# Autodesk Inventor assembly: panelsWithKerf
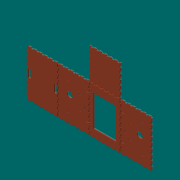
[picture p0: Inventor's stored thumbnail of the model, 180x180]
Saved by Autodesk Inventor 2016 SP2 (Build 200236200, 236)
## iProperties
Created: 2016-09-07
Part Number: panelsWithKerf
Document SubType Name: Assembly
Designer: sawaiz
Author: sawaiz
## Documents named in this file (8)
- C:\Users\sawaiz\OneDrive\projects\splitFlapDisplay\panelsWithKerf.iam
- C:\Users\sawaiz\oneDrive\projects\splitFlapDisplay\frame\front.ipt
- C:\Users\sawaiz\oneDrive\projects\splitFlapDisplay\frame\topBottomPanel.ipt
- C:\Users\sawaiz\oneDrive\projects\splitFlapDisplay\frame\leftSide.ipt
- C:\Users\sawaiz\oneDrive\projects\splitFlapDisplay\frame\rightSide.ipt
- C:\Users\sawaiz\oneDrive\projects\splitFlapDisplay\frame\back.ipt
- C:\Users\sawaiz\oneDrive\projects\splitFlapDisplay\panelsWithKerf.ipt
- C:\Users\sawaiz\OneDrive\projects\splitFlapDisplay\parameters.xlsx
## Components (6 placed, 6 different names)
1. front:1 — Flush:1, Flush:2, Flush:3, Flush:4, Flush:5, Flush:6, Flush:7, Flush:9, Mate:2, Mate:3, Mate:4
2. topBottomPanel:1 — Flush:3, Flush:5, Mate:3
3. leftSide:1 — Flush:2, Flush:7, Flush:8, Mate:1, Mate:2
4. rightSide:1 — Flush:4, Flush:6, Mate:4
5. back:1 — Flush:1, Flush:8, Mate:1
6. panelsWithKerf:1 — Flush:9
## Relationships (13: Flush 9, Mate 4)
- Flush:1: front:1 ↔ back:1
- Flush:2: front:1 ↔ leftSide:1
- Flush:3: front:1 ↔ topBottomPanel:1
- Flush:4: front:1 ↔ rightSide:1
- Flush:5: front:1 ↔ topBottomPanel:1
- Flush:6: front:1 ↔ rightSide:1
- Flush:7: front:1 ↔ leftSide:1
- Flush:8: leftSide:1 ↔ back:1
- Flush:9: front:1 ↔ panelsWithKerf:1
- Mate:1 (0.2 mm): leftSide:1 ↔ back:1
- Mate:2 (0.2 mm): front:1 ↔ leftSide:1
- Mate:3 (0.2 mm): front:1 ↔ topBottomPanel:1
- Mate:4 (0.2 mm): front:1 ↔ rightSide:1
## Named parameters: height = 180 mm, width = 120 mm, depth = 120 mm, materialThickness = 3.175 mm, laserKerf = 0.1 mm, spoolDiameter = 90 mm, cardPinDiameter = 3 mm, cardNumber = 40, centeralShaftDiameter = 8 mm, cardWidth = 85.6 mm, cardHeight = 53.98 mm, cardThickness = 0.76 mm, cardFillet = 2.88 mm, cardCutoutHeight = 20 mm, cardClearence = 0.5 mm, spoolHubDiameter = 20 mm, bearingOd = 22 mm, bearingWidth = 8 mm, axleHeight = 95 mm, nutTrapClearence = 2 mm, nutTrapwidth = 5.5 mm, nutTrapDepth = 2.5 mm, beltLength = 240 mm, magnetDiameter = 6 mm, magnetLength = 3 mm, magnetProtusion = 0.25 mm, notchWidth = 10 mm, spoolThickness = 5.588 mm
